# Autodesk Inventor assembly: wheel90mmwithbearing
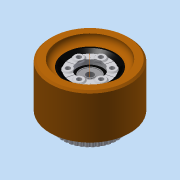
[picture p0: Inventor's stored thumbnail of the model, 180x180]
Saved by Autodesk Inventor 2014 SP1 (Build 180222100, 222)
## iProperties
Created: 2014-05-15
Part Number: wheel90mmwithbearing
Document SubType Name: Assembly
Designer: brent
Author: brent
## Documents named in this file (5)
- C:\Users\brent\Documents\electric-longboard\brent\wheel90mmwithbearing.iam
- C:\Users\brent\Documents\electric-longboard\brent\wheel90mm.ipt
- C:\Users\brent\Documents\electric-longboard\brent\608bearing.ipt
- C:\Users\brent\Documents\electric-longboard\brent\wheelinsertinner40t.ipt
- C:\Users\brent\Documents\electric-longboard\brent\wheelinsertouter.ipt
## Components (5 placed, 4 different names)
1. wheel90mm:1 — Insert:1, Insert:2, Mate:1, Mate:2, Mate:3, Mate:4
2. 608bearing:1 — Insert:2
3. 608bearing:2 — Insert:1
4. wheelinsertinner40t:1 — Mate:3, Mate:4
5. wheelinsertouter:1 — Mate:1, Mate:2
## Relationships (6: Mate 4, Insert 2)
- Insert:1: wheel90mm:1 ↔ 608bearing:2
- Insert:2: wheel90mm:1 ↔ 608bearing:1
- Mate:1 (-25.4 mm): wheel90mm:1 ↔ wheelinsertouter:1
- Mate:2: wheel90mm:1 ↔ wheelinsertouter:1
- Mate:3 (-64.008 mm): wheel90mm:1 ↔ wheelinsertinner40t:1
- Mate:4: wheel90mm:1 ↔ wheelinsertinner40t:1
